# Autodesk Inventor assembly: POM_T5_10
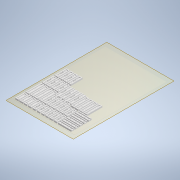
[picture p0: Inventor's stored thumbnail of the model, 180x180]
Saved by Autodesk Inventor 2020 (Build 240168000, 168)
## iProperties
Created: 2021-08-27
Part Number: POM_T5_10
Document SubType Name: Assembly
Designer: Masato
Author: Masato
## Documents named in this file (12)
- D:\GitHub\inventor\SUSTAINA-OP\Cam\POM_T5_10.iam
- D:\GitHub\inventor\SUSTAINA-OP\Cam\DisposableBoard.ipt
- D:\GitHub\inventor\SUSTAINA-OP\Jig\BackLink_diagonal_Jig.ipt
- D:\GitHub\inventor\SUSTAINA-OP\Jig\Foot_root_block_Jig.ipt
- D:\GitHub\inventor\SUSTAINA-OP\Jig\FrontLink_diagonal_Jig.ipt
- D:\GitHub\inventor\SUSTAINA-OP\Jig\Head_horn_frame_Jig.ipt
- D:\GitHub\inventor\SUSTAINA-OP\Jig\Leg_joint_yaw_frame_Jig.ipt
- D:\GitHub\inventor\SUSTAINA-OP\Jig\Shoulder_horn_frame_Jig.ipt
- D:\GitHub\inventor\SUSTAINA-OP\Jig\Trunk_chest_frame_Jig_1.ipt
- D:\GitHub\inventor\SUSTAINA-OP\Jig\Trunk_lower_side_frame_Jig.ipt
- D:\GitHub\inventor\SUSTAINA-OP\Jig\Trunk_chest_frame_Jig_2.ipt
- D:\GitHub\inventor\SUSTAINA-OP\Jig\UpperArm_diagonal_Jig.ipt
## Components (42 placed, 11 different names)
1. DisposableBoard:1 — メイト:2, メイト:1, フラッシュ:1, フラッシュ:2, メイト:4, メイト:5, メイト:6, メイト:10, メイト:11, メイト:13, メイト:15, メイト:17, メイト:20, メイト:21, メイト:23, メイト:25, メイト:26, メイト:28, メイト:29, メイト:32, メイト:35, メイト:37
2. BackLink_diagonal_Jig:2 — メイト:4, メイト:5, メイト:6, メイト:14
3. BackLink_diagonal_Jig:3
4. BackLink_diagonal_Jig:4
5. BackLink_diagonal_Jig:5 — メイト:16
6. Foot_root_block_Jig:1 — メイト:10, メイト:11, メイト:16, メイト:18
7. Foot_root_block_Jig:2
8. Foot_root_block_Jig:3
9. Foot_root_block_Jig:4 — メイト:22
10. FrontLink_diagonal_Jig:1 — メイト:13, メイト:14, メイト:15, メイト:27
11. FrontLink_diagonal_Jig:2
12. FrontLink_diagonal_Jig:3
13. FrontLink_diagonal_Jig:4 — メイト:19
14. Head_horn_frame_Jig:1 — メイト:17, メイト:18, メイト:19, メイト:30
15. Head_horn_frame_Jig:2
16. Head_horn_frame_Jig:3
17. Head_horn_frame_Jig:4
18. Trunk_chest_frame_Jig_1:2 — メイト:23, メイト:24, メイト:25
19. Trunk_chest_frame_Jig_1:3
20. Trunk_chest_frame_Jig_1:4
21. Trunk_chest_frame_Jig_1:5
22. Trunk_chest_frame_Jig_1:6 — メイト:33
23. Shoulder_horn_frame_Jig:1 — メイト:26, メイト:27, メイト:28, メイト:36
24. Shoulder_horn_frame_Jig:2
25. Shoulder_horn_frame_Jig:3
26. Shoulder_horn_frame_Jig:4 — メイト:31
27. Trunk_lower_side_frame_Jig:1 — メイト:29, メイト:30, メイト:31
28. Trunk_lower_side_frame_Jig:2
29. Trunk_lower_side_frame_Jig:3
30. Trunk_lower_side_frame_Jig:4 — メイト:34
31. Trunk_chest_frame_Jig_2:1 — メイト:32, メイト:33, メイト:34
32. Trunk_chest_frame_Jig_2:2
33. Trunk_chest_frame_Jig_2:3
34. Trunk_chest_frame_Jig_2:4
35. UpperArm_diagonal_Jig:1 — メイト:35, メイト:36, メイト:37
36. UpperArm_diagonal_Jig:2
37. UpperArm_diagonal_Jig:3
38. UpperArm_diagonal_Jig:4
39. Leg_joint_yaw_frame_Jig:1 — メイト:20, メイト:21, メイト:22
40. Leg_joint_yaw_frame_Jig:2 — メイト:24
41. Leg_joint_yaw_frame_Jig:3
42. Leg_joint_yaw_frame_Jig:4
## Component patterns: (4 elements, first: BackLink_diagonal_Jig:2), (4 elements, first: Foot_root_block_Jig:1), (4 elements, first: FrontLink_diagonal_Jig:1), (4 elements, first: Head_horn_frame_Jig:1), (2 elements), (5 elements, first: Trunk_chest_frame_Jig_1:2), (4 elements, first: Shoulder_horn_frame_Jig:1), (4 elements, first: Trunk_lower_side_frame_Jig:1), (4 elements, first: Trunk_chest_frame_Jig_2:1), (4 elements, first: UpperArm_diagonal_Jig:1), (2 elements, first: Leg_joint_yaw_frame_Jig:1), コンポーネント パターン 6:2 (2 elements)
## Relationships (34: Mate 32, Flush 2)
- メイト:2 [Mate]: DisposableBoard:1
- メイト:1 [Mate]: DisposableBoard:1
- フラッシュ:1 [Flush]: DisposableBoard:1
- フラッシュ:2 [Flush]: DisposableBoard:1
- メイト:4 [Mate]: DisposableBoard:1 ↔ BackLink_diagonal_Jig:2
- メイト:5 [Mate] (2.5 mm): DisposableBoard:1 ↔ BackLink_diagonal_Jig:2
- メイト:6 [Mate] (2.5 mm): DisposableBoard:1 ↔ BackLink_diagonal_Jig:2
- メイト:10 [Mate]: DisposableBoard:1 ↔ Foot_root_block_Jig:1
- メイト:11 [Mate] (2.5 mm): DisposableBoard:1 ↔ Foot_root_block_Jig:1
- メイト:13 [Mate]: DisposableBoard:1 ↔ FrontLink_diagonal_Jig:1
- メイト:14 [Mate] (3 mm): BackLink_diagonal_Jig:2 ↔ FrontLink_diagonal_Jig:1
- メイト:15 [Mate] (2.5 mm): DisposableBoard:1 ↔ FrontLink_diagonal_Jig:1
- メイト:16 [Mate] (3 mm): BackLink_diagonal_Jig:5 ↔ Foot_root_block_Jig:1
- メイト:17 [Mate]: DisposableBoard:1 ↔ Head_horn_frame_Jig:1
- メイト:18 [Mate] (3 mm): Foot_root_block_Jig:1 ↔ Head_horn_frame_Jig:1
- メイト:19 [Mate] (3 mm): FrontLink_diagonal_Jig:4 ↔ Head_horn_frame_Jig:1
- メイト:20 [Mate]: DisposableBoard:1 ↔ Leg_joint_yaw_frame_Jig:1
- メイト:21 [Mate] (2.5 mm): DisposableBoard:1 ↔ Leg_joint_yaw_frame_Jig:1
- メイト:22 [Mate] (3 mm): Foot_root_block_Jig:4 ↔ Leg_joint_yaw_frame_Jig:1
- メイト:23 [Mate]: DisposableBoard:1 ↔ Trunk_chest_frame_Jig_1:2
- メイト:24 [Mate] (3 mm): Trunk_chest_frame_Jig_1:2 ↔ Leg_joint_yaw_frame_Jig:2
- メイト:25 [Mate] (2.5 mm): DisposableBoard:1 ↔ Trunk_chest_frame_Jig_1:2
- メイト:26 [Mate]: DisposableBoard:1 ↔ Shoulder_horn_frame_Jig:1
- メイト:27 [Mate] (3 mm): FrontLink_diagonal_Jig:1 ↔ Shoulder_horn_frame_Jig:1
- メイト:28 [Mate] (2.5 mm): DisposableBoard:1 ↔ Shoulder_horn_frame_Jig:1
- メイト:29 [Mate]: DisposableBoard:1 ↔ Trunk_lower_side_frame_Jig:1
- メイト:30 [Mate] (3 mm): Head_horn_frame_Jig:1 ↔ Trunk_lower_side_frame_Jig:1
- メイト:31 [Mate] (3 mm): Shoulder_horn_frame_Jig:4 ↔ Trunk_lower_side_frame_Jig:1
- メイト:32 [Mate]: DisposableBoard:1 ↔ Trunk_chest_frame_Jig_2:1
- メイト:33 [Mate] (3 mm): Trunk_chest_frame_Jig_1:6 ↔ Trunk_chest_frame_Jig_2:1
- メイト:34 [Mate] (3 mm): Trunk_lower_side_frame_Jig:4 ↔ Trunk_chest_frame_Jig_2:1
- メイト:35 [Mate]: DisposableBoard:1 ↔ UpperArm_diagonal_Jig:1
- メイト:36 [Mate] (3 mm): Shoulder_horn_frame_Jig:1 ↔ UpperArm_diagonal_Jig:1
- メイト:37 [Mate] (2.5 mm): DisposableBoard:1 ↔ UpperArm_diagonal_Jig:1
